# Autodesk Inventor assembly: test
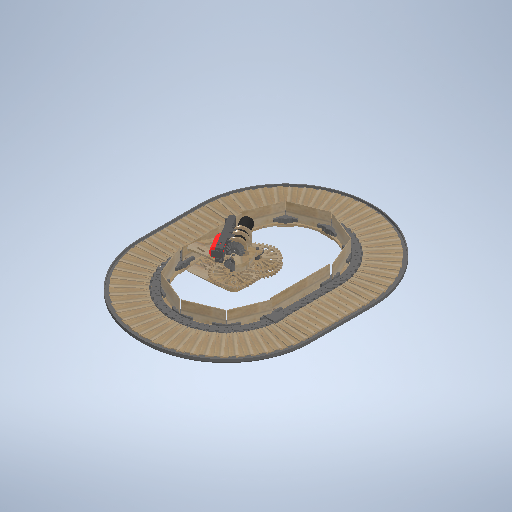
[picture p0: Inventor's stored thumbnail of the model, 512x512]
Saved by Autodesk Inventor 2026.1 (Build 301233020, 233B)
## iProperties
Created: 2025-09-27
Part Number: test
Document SubType Name: Assembly
Designer: hibik
Author: hibik
## Documents named in this file (4)
- C:\Users\hibik\Documents\Robomech\conveyer\All_body.iam
- C:\Users\hibik\Documents\Robomech\conveyer\liniar_module\Assy_linear_module.iam
- C:\Users\hibik\Documents\Robomech\conveyer\curve_module\Assy_curve_module.iam
- C:\Users\hibik\Documents\Robomech\conveyer\power_module\Assy_power_module.iam
## Components (11 placed, 3 different names)
1. Assy_linear_module:1 [sub-assembly] — メイト:1, メイト:2, フラッシュ:1, フラッシュ:11, 角度:1, 正接:1, 正接:2
2. Assy_curve_module:1 [sub-assembly] — メイト:1, メイト:2, フラッシュ:1, メイト:3, メイト:4, フラッシュ:2
3. Assy_curve_module:2 [sub-assembly] — メイト:3, メイト:4, フラッシュ:2, メイト:7, メイト:8, フラッシュ:4
4. Assy_curve_module:3 [sub-assembly] — メイト:7, メイト:8, フラッシュ:4
5. Assy_curve_module:4 [sub-assembly] — メイト:17, フラッシュ:9, メイト:18
6. Assy_curve_module:5 [sub-assembly] — メイト:19, メイト:20
7. Assy_curve_module:6 [sub-assembly]
8. Assy_curve_module:7 [sub-assembly]
9. Assy_curve_module:8 [sub-assembly] — フラッシュ:10
10. Assy_linear_module:2 [sub-assembly] — メイト:17, フラッシュ:9, メイト:18, フラッシュ:10, メイト:19, メイト:20
11. Assy_power_module:1 [sub-assembly] — フラッシュ:11, 角度:1, 正接:1, 正接:2
## Relationships (31: Mate 18, Flush 10, Tangent 2, Angle 1)
- メイト:1 [Mate]: Assy_linear_module:1 ↔ Assy_curve_module:1
- メイト:2 [Mate]: Assy_linear_module:1 ↔ Assy_curve_module:1
- フラッシュ:1 [Flush]: Assy_linear_module:1 ↔ Assy_curve_module:1
- メイト:3 [Mate]: Assy_curve_module:1 ↔ Assy_curve_module:2
- メイト:4 [Mate]: Assy_curve_module:1 ↔ Assy_curve_module:2
- フラッシュ:2 [Flush]: Assy_curve_module:1 ↔ Assy_curve_module:2
- [Mate]: Assy_curve_module:3 ↔ Assy_curve_module:4
- [Mate]: Assy_curve_module:3 ↔ Assy_curve_module:4
- [Flush]: Assy_curve_module:3 ↔ Assy_curve_module:4
- メイト:7 [Mate]: Assy_curve_module:2 ↔ Assy_curve_module:3
- メイト:8 [Mate]: Assy_curve_module:2 ↔ Assy_curve_module:3
- フラッシュ:4 [Flush]: Assy_curve_module:2 ↔ Assy_curve_module:3
- [Mate]: Assy_curve_module:5 ↔ Assy_curve_module:6
- [Mate]: Assy_curve_module:5 ↔ Assy_curve_module:6
- [Flush]: Assy_curve_module:5 ↔ Assy_curve_module:6
- [Mate]: Assy_curve_module:7 ↔ Assy_curve_module:8
- [Mate]: Assy_curve_module:7 ↔ Assy_curve_module:8
- [Flush]: Assy_curve_module:7 ↔ Assy_curve_module:8
- [Mate]: Assy_curve_module:6 ↔ Assy_curve_module:7
- [Mate]: Assy_curve_module:6 ↔ Assy_curve_module:7
- [Flush]: Assy_curve_module:6 ↔ Assy_curve_module:7
- メイト:17 [Mate]: Assy_curve_module:4 ↔ Assy_linear_module:2
- フラッシュ:9 [Flush]: Assy_curve_module:4 ↔ Assy_linear_module:2
- メイト:18 [Mate]: Assy_curve_module:4 ↔ Assy_linear_module:2
- フラッシュ:10 [Flush]: Assy_curve_module:8 ↔ Assy_linear_module:2
- メイト:19 [Mate]: Assy_curve_module:5 ↔ Assy_linear_module:2
- メイト:20 [Mate]: Assy_curve_module:5 ↔ Assy_linear_module:2
- フラッシュ:11 [Flush]: Assy_linear_module:1 ↔ Assy_power_module:1
- 角度:1 [Angle] (0 deg): Assy_linear_module:1 ↔ Assy_power_module:1
- 正接:1 [Tangent] (53 mm): Assy_linear_module:1 ↔ Assy_power_module:1
- 正接:2 [Tangent] (-15 mm): Assy_linear_module:1 ↔ Assy_power_module:1
## Named parameters: d62_d59 = 0 mm, d63_d60 = 0 mm, d64_d61 = 0 mm, d70_d59 = 0 mm, d71_d60 = 0 mm, d72_d61 = 0 mm, d73_d62_d59 = 0 mm, d74_d63_d60 = 0 mm, d75_d64_d61 = 0 mm, d76_d65 = 0 mm, d77_d66 = 0 mm, d78_d67 = 0 mm
